# Autodesk Inventor assembly: HatpHexa
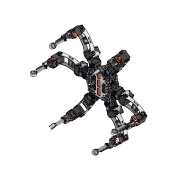
[picture p0: Inventor's stored thumbnail of the model, 180x180]
Saved by Autodesk Inventor 2021.2 (Build 252289000, 289)
## iProperties
Created: 2018-12-18
Part Number: HatpHexa
Material: 一般
Document SubType Name: Assembly
Designer: y6tada
Mass: 2014.19 g
Surface Area: 6659.5 cm^2
Volume: 1335.04 cm^3
Density: 1.50871 g/cm^3
Author: y6tada
## Documents named in this file (3)
- C:\Workspace\HaptHexa\Hardware\Inventor\00_000_HAPTHEXA_R3.iam
- C:\Workspace\HaptHexa\Hardware\Inventor\00_031_THORAX_R1.iam
- C:\Workspace\HaptHexa\Hardware\Inventor\00_002_SINGLE_LEG_R1.iam
## Components (7 placed, 2 different names)
1. 00_031_THORAX_R1:1 [sub-assembly] — Insert:1, Insert:2, Insert:3, Insert:4, Insert:5, Insert:6
2. 00_002_SINGLE_LEG_R1:1 [sub-assembly] — Insert:1
3. 00_002_SINGLE_LEG_R1:2 [sub-assembly] — Insert:2
4. 00_002_SINGLE_LEG_R1:3 [sub-assembly] — Insert:3
5. 00_002_SINGLE_LEG_R1:4 [sub-assembly] — Insert:4
6. 00_002_SINGLE_LEG_R1:5 [sub-assembly] — Insert:5
7. 00_002_SINGLE_LEG_R1:6 [sub-assembly] — Insert:6
## Relationships (6: Insert 6)
- Insert:1: 00_031_THORAX_R1:1 ↔ 00_002_SINGLE_LEG_R1:1
- Insert:2: 00_031_THORAX_R1:1 ↔ 00_002_SINGLE_LEG_R1:2
- Insert:3: 00_031_THORAX_R1:1 ↔ 00_002_SINGLE_LEG_R1:3
- Insert:4: 00_031_THORAX_R1:1 ↔ 00_002_SINGLE_LEG_R1:4
- Insert:5: 00_031_THORAX_R1:1 ↔ 00_002_SINGLE_LEG_R1:5
- Insert:6: 00_031_THORAX_R1:1 ↔ 00_002_SINGLE_LEG_R1:6
## Named parameters: femur_angle = 10 deg, tibia_angle = 80 deg
